# Autodesk Inventor assembly: SingleHeaterSiCMonofilamentAsembly
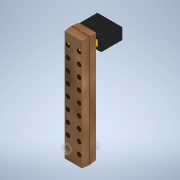
[picture p0: Inventor's stored thumbnail of the model, 180x180]
Saved by Autodesk Inventor 2021 (Build 250183000, 183)
## iProperties
Created: 2021-12-15
Part Number: SingleHeaterSiCMonofilamentAsembly
Document SubType Name: Assembly
Designer: Unit-005
Author: Unit-005
## Documents named in this file (6)
- C:\Users\Unit-005\Documents\Inventor\SiC_Monofilament_MicroheaterPrinthead\SingleHeaterSiCMonofilamentAsembly.iam
- C:\Users\Unit-005\Documents\Inventor\SiC_Monofilament_MicroheaterPrinthead\4mmSicFilament.ipt
- C:\Users\Unit-005\Documents\Inventor\SiC_Monofilament_MicroheaterPrinthead\VeroBoardLeadsSIngleHeater.ipt
- C:\Users\Unit-005\Documents\Inventor\SiC_Monofilament_MicroheaterPrinthead\VeroBoardLeadsSIngleHeater_MIR.ipt
- C:\Users\Unit-005\Documents\Inventor\SiC_Monofilament_MicroheaterPrinthead\din-84-slotted-cheese-head-screws-1.snapshot.2\DIN 84\M1 DIN 84.ipt
- C:\Users\Unit-005\Documents\Inventor\SiC_Monofilament_MicroheaterPrinthead\zl305-2s-2-54-5-58-2-5-5-1.snapshot.22\zl305-2s_p2-54_l5-58_w2-5_h5.ipt
## Components (6 placed, 5 different names)
1. 4mmSicFilament:1 — Mate:1, Tangent:1, Flush:1, Tangent:2, Flush:2
2. VeroBoardLeadsSIngleHeater:1 — Mate:1, Tangent:1, Flush:1, Mate:2, Mate:3, Mate:5, Mate:9
3. VeroBoardLeadsSIngleHeater_MIR:1 — Mate:4, Mate:5, Tangent:2, Flush:2, Mate:6, Mate:8
4. M1 DIN 84:1 — Mate:2, Mate:3
5. M1 DIN 84:2 — Mate:4, Mate:6
6. zl305-2s_p2-54_l5-58_w2-5_h5:1 — Mate:7, Mate:8, Mate:9
## Relationships (13: Mate 9, Tangent 2, Flush 2)
- Mate:1 (-0.0762 mm): 4mmSicFilament:1 ↔ VeroBoardLeadsSIngleHeater:1
- Tangent:1: 4mmSicFilament:1 ↔ VeroBoardLeadsSIngleHeater:1
- Flush:1: 4mmSicFilament:1 ↔ VeroBoardLeadsSIngleHeater:1
- Mate:2: VeroBoardLeadsSIngleHeater:1 ↔ M1 DIN 84:1
- Mate:3: VeroBoardLeadsSIngleHeater:1 ↔ M1 DIN 84:1
- Mate:4: VeroBoardLeadsSIngleHeater_MIR:1 ↔ M1 DIN 84:2
- Mate:5: VeroBoardLeadsSIngleHeater:1 ↔ VeroBoardLeadsSIngleHeater_MIR:1
- Tangent:2: 4mmSicFilament:1 ↔ VeroBoardLeadsSIngleHeater_MIR:1
- Flush:2: 4mmSicFilament:1 ↔ VeroBoardLeadsSIngleHeater_MIR:1
- Mate:6: VeroBoardLeadsSIngleHeater_MIR:1 ↔ M1 DIN 84:2
- Mate:7: zl305-2s_p2-54_l5-58_w2-5_h5:1
- Mate:8: VeroBoardLeadsSIngleHeater_MIR:1 ↔ zl305-2s_p2-54_l5-58_w2-5_h5:1
- Mate:9: VeroBoardLeadsSIngleHeater:1 ↔ zl305-2s_p2-54_l5-58_w2-5_h5:1
